# Autodesk Inventor assembly: GP10-100
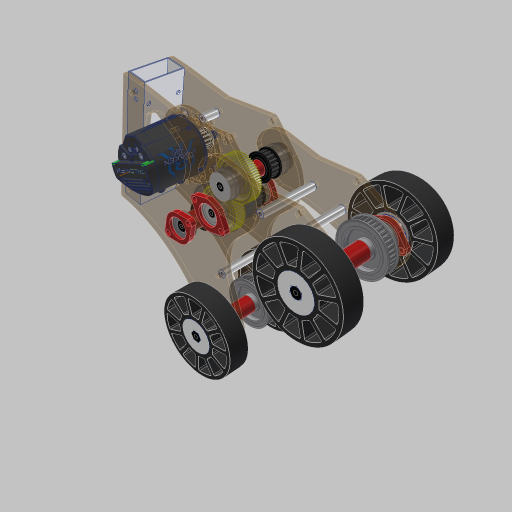
[picture p0: Inventor's stored thumbnail of the model, 512x512]
Saved by Autodesk Inventor 2023.5 (Build 275446000, 446)
## iProperties
Created: 2025-03-20
Part Number: GP10-100
Document SubType Name: Assembly
Designer: slick
Author: slick
## Documents named in this file (34)
- C:\Users\slick\OneDrive\Desktop\2025-ReefScape---CAD\Gripper\GP10\GP10-100.iam
- C:\Users\slick\OneDrive\Desktop\2025-ReefScape---CAD\Gripper\GP10\GP10-001.ipt
- C:\Users\slick\OneDrive\Desktop\2025-ReefScape---CAD\Gripper\GP10\GP10-002.ipt
- C:\Users\slick\OneDrive\Desktop\2025-ReefScape---CAD\Gripper\GP10\GP10-003.ipt
- C:\Users\slick\OneDrive\Desktop\2025-ReefScape---CAD\COMMON PARTS\BEARINGS\13_75mm_1_2_ThunderHex_ID_x_1_125_OD_x_0_313_WD_Flanged_Bearing_217-4006_MIR.ipt
- C:\Users\slick\OneDrive\Desktop\2025-ReefScape---CAD\Gripper\GP10\GP10-005.ipt
- C:\Users\slick\OneDrive\Desktop\2025-ReefScape---CAD\COMMON PARTS\BEARINGS\0_500_ID_x_1_125_OD_x_0_313_WD_Flanged_Bearing_217-2731.ipt
- C:\Users\slick\OneDrive\Desktop\2025-ReefScape---CAD\COMMON PARTS\BEARINGS\Bearing Retainer\Retainer.ipt
- C:\Users\slick\OneDrive\Desktop\2025-ReefScape---CAD\Gripper\GP10\GP10-007.ipt
- C:\Users\slick\OneDrive\Desktop\2025-ReefScape---CAD\COMMON PARTS\WHEELS\am-3480 4IN 500Hex Bore Compliant Wheel REV2 (1).iam
- C:\Users\slick\OneDrive\Desktop\2025-ReefScape---CAD\COMMON PARTS\BEARINGS\0_375_ID_x_1_125_OD_x_0_313_WD_Flanged_Bearing_217-2732.ipt
- C:\Users\slick\OneDrive\Desktop\2025-ReefScape---CAD\Gripper\GP10\GP10-008.ipt
- C:\Users\slick\OneDrive\Desktop\2025-ReefScape---CAD\Gripper\GP10\GP10-009.ipt
- C:\Users\slick\OneDrive\Desktop\2025-ReefScape---CAD\Gripper\GP10\GP10-010.ipt
- C:\Users\slick\OneDrive\Desktop\2025-ReefScape---CAD\Gripper\GP10\GP10-004.ipt
- C:\Users\slick\OneDrive\Desktop\2025-ReefScape---CAD\COMMON PARTS\MOTORS\Kracken X60WCP-0940 (1).ipt
- C:\Users\slick\OneDrive\Desktop\2025-ReefScape---CAD\COMMON PARTS\PULLEYS\htd\WCP-1017 (1)\WCP-1017 (1).ipt
- C:\Users\slick\OneDrive\Desktop\2025-ReefScape---CAD\COMMON PARTS\PULLEYS\htd\36t_x_9mm_Wide_Double_Flange_Aluminum_Pulley_HTD_5mm_1_2_Hex_Bore_217-3231.ipt
- C:\Users\slick\OneDrive\Desktop\2025-ReefScape---CAD\COMMON PARTS\PULLEYS\htd\18t_x_9mm_Wide_Double_Flange_Aluminum_Pulley_HTD_5mm_1_2_Hex_Bore_217-3225.ipt
- C:\Users\slick\OneDrive\Desktop\2025-ReefScape---CAD\Gripper\GP10\GP10-011.ipt
- C:\Users\slick\OneDrive\Desktop\2025-ReefScape---CAD\Gripper\GP10\GP10-012.ipt
- C:\Users\slick\OneDrive\Desktop\2025-ReefScape---CAD\COMMON PARTS\GEARS\32 dp gear\60t_Aluminum_Spur_Gear_32_DP_3_8_Hex_Bore_217-5863.ipt
- C:\Users\slick\OneDrive\Desktop\2025-ReefScape---CAD\COMMON PARTS\PULLEYS\htd\24t_x_9mm_Wide_Double_Flange_Aluminum_Pulley_HTD_5mm_1_2_Hex_Bore_217-3227.ipt
- C:\Users\slick\OneDrive\Desktop\2025-ReefScape---CAD\Gripper\GP10\Spacers\GP-SP-001.ipt
- C:\Users\slick\OneDrive\Desktop\2025-ReefScape---CAD\Gripper\GP10\Spacers\GP-SP-002.ipt
- C:\Users\slick\OneDrive\Desktop\2025-ReefScape---CAD\Gripper\GP10\Spacers\GP-SP-003.ipt
- C:\Users\slick\OneDrive\Desktop\2025-ReefScape---CAD\Gripper\GP10\Spacers\GP-SP-004.ipt
- C:\Users\slick\OneDrive\Desktop\2025-ReefScape---CAD\Gripper\GP10\Spacers\GP-SP-005.ipt
- C:\Users\slick\OneDrive\Desktop\2025-ReefScape---CAD\Gripper\GP10\Spacers\GP-SP-006.ipt
- C:\Users\slick\OneDrive\Desktop\2025-ReefScape---CAD\Gripper\GP10\Spacers\GP-SP-007.ipt
- C:\Users\slick\OneDrive\Desktop\2025-ReefScape---CAD\Gripper\GP10\Spacers\GP-SP-008.ipt
- C:\Users\slick\OneDrive\Desktop\2025-ReefScape---CAD\Gripper\GP10\Spacers\GP-SP-009.ipt
- C:\Users\slick\OneDrive\Desktop\2025-ReefScape---CAD\Gripper\GP10\GP10-013.ipt
- C:\Users\slick\OneDrive\Desktop\2025-ReefScape---CAD\Gripper\GP10\GP10-014.ipt
## Components (70 placed, 33 different names)
1. GP10-001:1 — Mate:1, Angle:1, Mate:3, Flush:1, Mate:5, Insert:4, Insert:9, Insert:10, Insert:21, Insert:24, Insert:25, Insert:28, Insert:29, Insert:30, Insert:31, Mate:22, Mate:24, Insert:36, Insert:38, Insert:41, Insert:42, Insert:47, Insert:48, Mate:52, Mate:53, Mate:62
2. GP10-002:1 — Mate:1, Angle:1, Mate:3, Mate:7, Insert:3, Insert:16, Insert:17, Insert:37, Mate:64
3. GP10-003:1 — Flush:1, Mate:5, Mate:6, Insert:1, Insert:11, Insert:22, Insert:26, Insert:27, Insert:35, Insert:39, Insert:43, Insert:44, Insert:45, Insert:46, Mate:37, Mate:47, Mate:49, Mate:68, Insert:52
4. GP10-002:2 — Mate:6, Mate:7, Insert:2, Insert:18, Insert:19, Insert:40, Insert:50, Insert:51
5. GP10-005:1 — Insert:9, Insert:10, Insert:11
6. Retainer:1 — Insert:16, Insert:17
7. Retainer:2 — Insert:18, Insert:19, Mate:14
8. GP10-007:1 — Mate:11, Mate:12, Flush:3, Mate:13, Flush:4, Mate:44, Mate:69, Mate:73, Mate:75
9. am-3480 4IN 500Hex Bore Compliant Wheel REV2 (1):1 [sub-assembly] — Mate:12, Flush:3, Mate:63
10. am-3480 4IN 500Hex Bore Compliant Wheel REV2 (1):2 [sub-assembly] — Mate:13, Flush:4, Mate:14
11. GP10-008:2 — Mate:16, Flush:6, Mate:35, Mate:38, Mate:41, Mate:46, Mate:57, Mate:59
12. GP10-009:1 — Mate:17, Mate:18, Flush:7, Flush:8, Mate:19, Mate:43, Mate:51, Mate:65, Mate:77, Mate:79
13. am-3480 4IN 500Hex Bore Compliant Wheel REV2 (1):3 [sub-assembly] — Mate:18, Flush:7
14. am-3480 4IN 500Hex Bore Compliant Wheel REV2 (1):4 [sub-assembly] — Flush:8, Mate:19, Mate:20
15. Retainer:3 — Insert:24, Insert:25
16. Retainer:4 — Insert:26, Insert:27, Mate:20
17. GP10-010:1 — Insert:28, Insert:32
18. GP10-010:2 — Insert:29
19. GP10-010:3 — Insert:30
20. GP10-010:4 — Insert:31, Insert:33
21. GP10-004:1 — Insert:32, Insert:33, Mate:21, Insert:34
22. Kracken X60WCP-0940 (1):1 — Mate:21, Mate:22, Insert:34, Mate:23
23. WCP-1017 (1):1 — Mate:23, Mate:24
24. 36t_x_9mm_Wide_Double_Flange_Aluminum_Pulley_HTD_5mm_1_2_Hex_Bore_217-3231:1 — Mate:28, Mate:32, Mate:33, Mate:56
25. 18t_x_9mm_Wide_Double_Flange_Aluminum_Pulley_HTD_5mm_1_2_Hex_Bore_217-3225:1 — Mate:28, Flush:12, Mate:54
26. 0_500_ID_x_1_125_OD_x_0_313_WD_Flanged_Bearing_217-2731:1 — Insert:35, Mate:31, Flush:9, Mate:32, Mate:54, Mate:55, Mate:67
27. Retainer:5 — Insert:43, Insert:44
28. Retainer:6 — Insert:41, Insert:42
29. Retainer:7 — Insert:47, Insert:48
30. Retainer:8 — Insert:45, Insert:46
31. GP10-011:1 — Mate:31, Flush:9
32. GP10-012:1 — Mate:34, Flush:10, Mate:36, Mate:40, Mate:48, Mate:61, Mate:71
33. 60t_Aluminum_Spur_Gear_32_DP_3_8_Hex_Bore_217-5863:1 — Mate:36, Flush:11, Mate:72
34. 60t_Aluminum_Spur_Gear_32_DP_3_8_Hex_Bore_217-5863:2 — Mate:35, Flush:11, Mate:37, Mate:58
35. 24t_x_9mm_Wide_Double_Flange_Aluminum_Pulley_HTD_5mm_1_2_Hex_Bore_217-3227:1 — Mate:38, Flush:12, Mate:60
36. 18t_x_9mm_Wide_Double_Flange_Aluminum_Pulley_HTD_5mm_1_2_Hex_Bore_217-3225:2 — Mate:39, Mate:40, Flush:13
37. 18t_x_9mm_Wide_Double_Flange_Aluminum_Pulley_HTD_5mm_1_2_Hex_Bore_217-3225:3 — Mate:41, Mate:42
38. 36t_x_9mm_Wide_Double_Flange_Aluminum_Pulley_HTD_5mm_1_2_Hex_Bore_217-3231:2 — Mate:43, Mate:45, Mate:66
39. 36t_x_9mm_Wide_Double_Flange_Aluminum_Pulley_HTD_5mm_1_2_Hex_Bore_217-3231:3 — Mate:44, Flush:13, Mate:70
40. GP10-013:1 — Insert:52
41. GP10-014:1 — Insert:51
42. GP10-014:2 — Insert:50
43. 0_375_ID_x_1_125_OD_x_0_313_WD_Flanged_Bearing_217-2732:3 — Insert:21, Mate:16, Flush:6, Mate:42
44. 0_375_ID_x_1_125_OD_x_0_313_WD_Flanged_Bearing_217-2732:4 — Insert:22
45. 0_500_ID_x_1_125_OD_x_0_313_WD_Flanged_Bearing_217-2731:2 — Insert:36, Mate:33, Mate:50
46. 0_375_ID_x_1_125_OD_x_0_313_WD_Flanged_Bearing_217-2732:5 — Insert:37, Mate:29
47. 0_375_ID_x_1_125_OD_x_0_313_WD_Flanged_Bearing_217-2732:6 — Insert:38, Mate:29, Mate:39
48. 0_375_ID_x_1_125_OD_x_0_313_WD_Flanged_Bearing_217-2732:7 — Insert:40, Mate:30, Mate:34, Flush:10
49. 0_375_ID_x_1_125_OD_x_0_313_WD_Flanged_Bearing_217-2732:8 — Insert:39, Mate:30
50. 13_75mm_1_2_ThunderHex_ID_x_1_125_OD_x_0_313_WD_Flanged_Bearing_217-4006_MIR:1 — Insert:3, Mate:11, Mate:74
51. 13_75mm_1_2_ThunderHex_ID_x_1_125_OD_x_0_313_WD_Flanged_Bearing_217-4006_MIR:2 — Insert:2, Mate:76
52. 13_75mm_1_2_ThunderHex_ID_x_1_125_OD_x_0_313_WD_Flanged_Bearing_217-4006_MIR:3 — Insert:1, Mate:78
53. 13_75mm_1_2_ThunderHex_ID_x_1_125_OD_x_0_313_WD_Flanged_Bearing_217-4006_MIR:4 — Insert:4, Mate:17, Mate:45, Mate:80
54. GP-SP-009:1 — Mate:77, Mate:78
55. GP-SP-009:2 — Mate:79, Mate:80
56. GP-SP-009:3 — Mate:75, Mate:76
57. GP-SP-009:4 — Mate:73, Mate:74
58. GP-SP-008:1 — Mate:71, Mate:72
59. GP-SP-007:1 — Mate:69, Mate:70
60. GP-SP-006:1 — Mate:67, Mate:68
61. GP-SP-005:1 — Mate:65, Mate:66
62. GP-SP-004:1 — Mate:57, Mate:58
63. GP-SP-004:2 — Mate:59, Mate:60
64. GP-SP-003:1 — Mate:63, Mate:64
65. GP-SP-002:3 — Mate:55, Mate:56
66. GP-SP-002:1 — Mate:50, Mate:52
67. GP-SP-002:2 — Mate:51, Mate:53
68. GP-SP-001:1 — Mate:48, Mate:49
69. GP-SP-001:2 — Mate:46, Mate:47
70. GP-SP-001:3 — Mate:61, Mate:62
## Relationships (124: Mate 71, Insert 41, Flush 11, Angle 1)
- Mate:1: GP10-001:1 ↔ GP10-002:1
- Angle:1 (0 deg): GP10-001:1 ↔ GP10-002:1
- Mate:3: GP10-001:1 ↔ GP10-002:1
- Flush:1: GP10-001:1 ↔ GP10-003:1
- Mate:5: GP10-001:1 ↔ GP10-003:1
- Mate:6: GP10-003:1 ↔ GP10-002:2
- Mate:7: GP10-002:1 ↔ GP10-002:2
- Insert:1: GP10-003:1 ↔ 13_75mm_1_2_ThunderHex_ID_x_1_125_OD_x_0_313_WD_Flanged_Bearing_217-4006_MIR:3
- Insert:2: GP10-002:2 ↔ 13_75mm_1_2_ThunderHex_ID_x_1_125_OD_x_0_313_WD_Flanged_Bearing_217-4006_MIR:2
- Insert:3: GP10-002:1 ↔ 13_75mm_1_2_ThunderHex_ID_x_1_125_OD_x_0_313_WD_Flanged_Bearing_217-4006_MIR:1
- Insert:4: GP10-001:1 ↔ 13_75mm_1_2_ThunderHex_ID_x_1_125_OD_x_0_313_WD_Flanged_Bearing_217-4006_MIR:4
- Insert:9: GP10-001:1 ↔ GP10-005:1
- Insert:10: GP10-001:1 ↔ GP10-005:1
- Insert:11: GP10-003:1 ↔ GP10-005:1
- Insert:16: GP10-002:1 ↔ Retainer:1
- Insert:17: GP10-002:1 ↔ Retainer:1
- Insert:18: GP10-002:2 ↔ Retainer:2
- Insert:19: GP10-002:2 ↔ Retainer:2
- Mate:11: GP10-007:1 ↔ 13_75mm_1_2_ThunderHex_ID_x_1_125_OD_x_0_313_WD_Flanged_Bearing_217-4006_MIR:1
- Mate:12: GP10-007:1 ↔ am-3480 4IN 500Hex Bore Compliant Wheel REV2 (1):1
- Flush:3: GP10-007:1 ↔ am-3480 4IN 500Hex Bore Compliant Wheel REV2 (1):1
- Mate:13: GP10-007:1 ↔ am-3480 4IN 500Hex Bore Compliant Wheel REV2 (1):2
- Flush:4: GP10-007:1 ↔ am-3480 4IN 500Hex Bore Compliant Wheel REV2 (1):2
- Mate:14 (3.175 mm): Retainer:2 ↔ am-3480 4IN 500Hex Bore Compliant Wheel REV2 (1):2
- Insert:21: GP10-001:1 ↔ 0_375_ID_x_1_125_OD_x_0_313_WD_Flanged_Bearing_217-2732:3
- Insert:22: GP10-003:1 ↔ 0_375_ID_x_1_125_OD_x_0_313_WD_Flanged_Bearing_217-2732:4
- Mate:16: GP10-008:2 ↔ 0_375_ID_x_1_125_OD_x_0_313_WD_Flanged_Bearing_217-2732:3
- Flush:6: GP10-008:2 ↔ 0_375_ID_x_1_125_OD_x_0_313_WD_Flanged_Bearing_217-2732:3
- Mate:17: GP10-009:1 ↔ 13_75mm_1_2_ThunderHex_ID_x_1_125_OD_x_0_313_WD_Flanged_Bearing_217-4006_MIR:4
- Mate:18: GP10-009:1 ↔ am-3480 4IN 500Hex Bore Compliant Wheel REV2 (1):3
- Flush:7: GP10-009:1 ↔ am-3480 4IN 500Hex Bore Compliant Wheel REV2 (1):3
- Flush:8: GP10-009:1 ↔ am-3480 4IN 500Hex Bore Compliant Wheel REV2 (1):4
- Mate:19: GP10-009:1 ↔ am-3480 4IN 500Hex Bore Compliant Wheel REV2 (1):4
- Insert:24: GP10-001:1 ↔ Retainer:3
- Insert:25: GP10-001:1 ↔ Retainer:3
- Insert:26: GP10-003:1 ↔ Retainer:4
- Insert:27: GP10-003:1 ↔ Retainer:4
- Mate:20 (3.175 mm): am-3480 4IN 500Hex Bore Compliant Wheel REV2 (1):4 ↔ Retainer:4
- Insert:28: GP10-001:1 ↔ GP10-010:1
- Insert:29: GP10-001:1 ↔ GP10-010:2
- Insert:30: GP10-001:1 ↔ GP10-010:3
- Insert:31: GP10-001:1 ↔ GP10-010:4
- Insert:32: GP10-010:1 ↔ GP10-004:1
- Insert:33: GP10-010:4 ↔ GP10-004:1
- Mate:21: GP10-004:1 ↔ Kracken X60WCP-0940 (1):1
- Mate:22: GP10-001:1 ↔ Kracken X60WCP-0940 (1):1
- Insert:34: GP10-004:1 ↔ Kracken X60WCP-0940 (1):1
- Mate:23: Kracken X60WCP-0940 (1):1 ↔ WCP-1017 (1):1
- Mate:24: GP10-001:1 ↔ WCP-1017 (1):1
- Mate:28 (1.5875 mm): 36t_x_9mm_Wide_Double_Flange_Aluminum_Pulley_HTD_5mm_1_2_Hex_Bore_217-3231:1 ↔ 18t_x_9mm_Wide_Double_Flange_Aluminum_Pulley_HTD_5mm_1_2_Hex_Bore_217-3225:1
- Insert:35: GP10-003:1 ↔ 0_500_ID_x_1_125_OD_x_0_313_WD_Flanged_Bearing_217-2731:1
- Insert:36: GP10-001:1 ↔ 0_500_ID_x_1_125_OD_x_0_313_WD_Flanged_Bearing_217-2731:2
- Insert:37: GP10-002:1 ↔ 0_375_ID_x_1_125_OD_x_0_313_WD_Flanged_Bearing_217-2732:5
- Insert:38: GP10-001:1 ↔ 0_375_ID_x_1_125_OD_x_0_313_WD_Flanged_Bearing_217-2732:6
- Insert:39: GP10-003:1 ↔ 0_375_ID_x_1_125_OD_x_0_313_WD_Flanged_Bearing_217-2732:8
- Insert:40: GP10-002:2 ↔ 0_375_ID_x_1_125_OD_x_0_313_WD_Flanged_Bearing_217-2732:7
- Mate:29: 0_375_ID_x_1_125_OD_x_0_313_WD_Flanged_Bearing_217-2732:5 ↔ 0_375_ID_x_1_125_OD_x_0_313_WD_Flanged_Bearing_217-2732:6
- Mate:30: 0_375_ID_x_1_125_OD_x_0_313_WD_Flanged_Bearing_217-2732:7 ↔ 0_375_ID_x_1_125_OD_x_0_313_WD_Flanged_Bearing_217-2732:8
- Insert:41: GP10-001:1 ↔ Retainer:6
- Insert:42: GP10-001:1 ↔ Retainer:6
- Insert:43: GP10-003:1 ↔ Retainer:5
- Insert:44: GP10-003:1 ↔ Retainer:5
- Insert:45: GP10-003:1 ↔ Retainer:8
- Insert:46: GP10-003:1 ↔ Retainer:8
- Insert:47: GP10-001:1 ↔ Retainer:7
- Insert:48: GP10-001:1 ↔ Retainer:7
- Mate:31: 0_500_ID_x_1_125_OD_x_0_313_WD_Flanged_Bearing_217-2731:1 ↔ GP10-011:1
- Flush:9: 0_500_ID_x_1_125_OD_x_0_313_WD_Flanged_Bearing_217-2731:1 ↔ GP10-011:1
- Mate:32: 36t_x_9mm_Wide_Double_Flange_Aluminum_Pulley_HTD_5mm_1_2_Hex_Bore_217-3231:1 ↔ 0_500_ID_x_1_125_OD_x_0_313_WD_Flanged_Bearing_217-2731:1
- Mate:33 (1.5875 mm): 36t_x_9mm_Wide_Double_Flange_Aluminum_Pulley_HTD_5mm_1_2_Hex_Bore_217-3231:1 ↔ 0_500_ID_x_1_125_OD_x_0_313_WD_Flanged_Bearing_217-2731:2
- Mate:34: GP10-012:1 ↔ 0_375_ID_x_1_125_OD_x_0_313_WD_Flanged_Bearing_217-2732:7
- Flush:10: GP10-012:1 ↔ 0_375_ID_x_1_125_OD_x_0_313_WD_Flanged_Bearing_217-2732:7
- Mate:35: GP10-008:2 ↔ 60t_Aluminum_Spur_Gear_32_DP_3_8_Hex_Bore_217-5863:2
- Mate:36: GP10-012:1 ↔ 60t_Aluminum_Spur_Gear_32_DP_3_8_Hex_Bore_217-5863:1
- Flush:11: 60t_Aluminum_Spur_Gear_32_DP_3_8_Hex_Bore_217-5863:1 ↔ 60t_Aluminum_Spur_Gear_32_DP_3_8_Hex_Bore_217-5863:2
- Mate:37 (1.5875 mm): GP10-003:1 ↔ 60t_Aluminum_Spur_Gear_32_DP_3_8_Hex_Bore_217-5863:2
- Mate:38: GP10-008:2 ↔ 24t_x_9mm_Wide_Double_Flange_Aluminum_Pulley_HTD_5mm_1_2_Hex_Bore_217-3227:1
- Flush:12: 18t_x_9mm_Wide_Double_Flange_Aluminum_Pulley_HTD_5mm_1_2_Hex_Bore_217-3225:1 ↔ 24t_x_9mm_Wide_Double_Flange_Aluminum_Pulley_HTD_5mm_1_2_Hex_Bore_217-3227:1
- Mate:39 (1.5875 mm): 18t_x_9mm_Wide_Double_Flange_Aluminum_Pulley_HTD_5mm_1_2_Hex_Bore_217-3225:2 ↔ 0_375_ID_x_1_125_OD_x_0_313_WD_Flanged_Bearing_217-2732:6
- Mate:40: GP10-012:1 ↔ 18t_x_9mm_Wide_Double_Flange_Aluminum_Pulley_HTD_5mm_1_2_Hex_Bore_217-3225:2
- Mate:41: GP10-008:2 ↔ 18t_x_9mm_Wide_Double_Flange_Aluminum_Pulley_HTD_5mm_1_2_Hex_Bore_217-3225:3
- Mate:42: 18t_x_9mm_Wide_Double_Flange_Aluminum_Pulley_HTD_5mm_1_2_Hex_Bore_217-3225:3 ↔ 0_375_ID_x_1_125_OD_x_0_313_WD_Flanged_Bearing_217-2732:3
- Mate:43: GP10-009:1 ↔ 36t_x_9mm_Wide_Double_Flange_Aluminum_Pulley_HTD_5mm_1_2_Hex_Bore_217-3231:2
- Mate:44: GP10-007:1 ↔ 36t_x_9mm_Wide_Double_Flange_Aluminum_Pulley_HTD_5mm_1_2_Hex_Bore_217-3231:3
- Mate:45 (1.5875 mm): 36t_x_9mm_Wide_Double_Flange_Aluminum_Pulley_HTD_5mm_1_2_Hex_Bore_217-3231:2 ↔ 13_75mm_1_2_ThunderHex_ID_x_1_125_OD_x_0_313_WD_Flanged_Bearing_217-4006_MIR:4
- Flush:13: 18t_x_9mm_Wide_Double_Flange_Aluminum_Pulley_HTD_5mm_1_2_Hex_Bore_217-3225:2 ↔ 36t_x_9mm_Wide_Double_Flange_Aluminum_Pulley_HTD_5mm_1_2_Hex_Bore_217-3231:3
- Mate:46: GP10-008:2 ↔ GP-SP-001:2
- Mate:47: GP10-003:1 ↔ GP-SP-001:2
- Mate:48: GP10-012:1 ↔ GP-SP-001:1
- Mate:49: GP10-003:1 ↔ GP-SP-001:1
- Mate:50: 0_500_ID_x_1_125_OD_x_0_313_WD_Flanged_Bearing_217-2731:2 ↔ GP-SP-002:1
- Mate:51: GP10-009:1 ↔ GP-SP-002:2
- Mate:52: GP10-001:1 ↔ GP-SP-002:1
- Mate:53: GP10-001:1 ↔ GP-SP-002:2
- Mate:54: 18t_x_9mm_Wide_Double_Flange_Aluminum_Pulley_HTD_5mm_1_2_Hex_Bore_217-3225:1 ↔ 0_500_ID_x_1_125_OD_x_0_313_WD_Flanged_Bearing_217-2731:1
- Mate:55: 0_500_ID_x_1_125_OD_x_0_313_WD_Flanged_Bearing_217-2731:1 ↔ GP-SP-002:3
- Mate:56: 36t_x_9mm_Wide_Double_Flange_Aluminum_Pulley_HTD_5mm_1_2_Hex_Bore_217-3231:1 ↔ GP-SP-002:3
- Mate:57: GP10-008:2 ↔ GP-SP-004:1
- Mate:58: 60t_Aluminum_Spur_Gear_32_DP_3_8_Hex_Bore_217-5863:2 ↔ GP-SP-004:1
- Mate:59: GP10-008:2 ↔ GP-SP-004:2
- Mate:60: 24t_x_9mm_Wide_Double_Flange_Aluminum_Pulley_HTD_5mm_1_2_Hex_Bore_217-3227:1 ↔ GP-SP-004:2
- Mate:61: GP10-012:1 ↔ GP-SP-001:3
- Mate:62: GP10-001:1 ↔ GP-SP-001:3
- Mate:63: am-3480 4IN 500Hex Bore Compliant Wheel REV2 (1):1 ↔ GP-SP-003:1
- Mate:64: GP10-002:1 ↔ GP-SP-003:1
- Mate:65: GP10-009:1 ↔ GP-SP-005:1
- Mate:66: 36t_x_9mm_Wide_Double_Flange_Aluminum_Pulley_HTD_5mm_1_2_Hex_Bore_217-3231:2 ↔ GP-SP-005:1
- Mate:67: 0_500_ID_x_1_125_OD_x_0_313_WD_Flanged_Bearing_217-2731:1 ↔ GP-SP-006:1
- Mate:68: GP10-003:1 ↔ GP-SP-006:1
- Mate:69: GP10-007:1 ↔ GP-SP-007:1
- Mate:70: 36t_x_9mm_Wide_Double_Flange_Aluminum_Pulley_HTD_5mm_1_2_Hex_Bore_217-3231:3 ↔ GP-SP-007:1
- Mate:71: GP10-012:1 ↔ GP-SP-008:1
- Mate:72: 60t_Aluminum_Spur_Gear_32_DP_3_8_Hex_Bore_217-5863:1 ↔ GP-SP-008:1
- Mate:73: GP10-007:1 ↔ GP-SP-009:4
- Mate:74: 13_75mm_1_2_ThunderHex_ID_x_1_125_OD_x_0_313_WD_Flanged_Bearing_217-4006_MIR:1 ↔ GP-SP-009:4
- Mate:75: GP10-007:1 ↔ GP-SP-009:3
- Mate:76: 13_75mm_1_2_ThunderHex_ID_x_1_125_OD_x_0_313_WD_Flanged_Bearing_217-4006_MIR:2 ↔ GP-SP-009:3
- Mate:77: GP10-009:1 ↔ GP-SP-009:1
- Mate:78: 13_75mm_1_2_ThunderHex_ID_x_1_125_OD_x_0_313_WD_Flanged_Bearing_217-4006_MIR:3 ↔ GP-SP-009:1
- Mate:79: GP10-009:1 ↔ GP-SP-009:2
- Mate:80: 13_75mm_1_2_ThunderHex_ID_x_1_125_OD_x_0_313_WD_Flanged_Bearing_217-4006_MIR:4 ↔ GP-SP-009:2
- Insert:50: GP10-002:2 ↔ GP10-014:2
- Insert:51: GP10-002:2 ↔ GP10-014:1
- Insert:52: GP10-003:1 ↔ GP10-013:1
